# Autodesk Inventor assembly: 99535c01
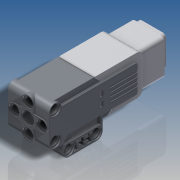
[picture p0: Inventor's stored thumbnail of the model, 180x180]
Saved by Autodesk Inventor 2016 SP2 (Build 200236200, 236)
## iProperties
Created: 2015-09-02
Part Number: 99535c01
Document SubType Name: Assembly
Designer: D. Kohfeld
Mass: 14.5508 g
Surface Area: 210.492 cm^2
Volume: 13.7272 cm^3
Density: 1.06 g/cm^3
Author: D. Kohfeld
## Documents named in this file (5)
- A:\LEGO Pieces\EV3\99535c01.iam
- A:\LEGO Pieces\EV3\99534-White.ipt
- A:\LEGO Pieces\EV3\54732b-LtBluishGray.ipt
- A:\LEGO Pieces\EV3\99542-MilkyWhite.ipt
- A:\LEGO Pieces\EV3\99535-LtBluishGray.ipt
## Components (4 placed, 4 different names)
1. 99534-White:1 — Mate:1, Mate:2, Flush:1, Flush:2, Flush:3, Mate:3
2. 54732b-LtBluishGray:1 — Mate:1, Mate:2, Flush:1
3. 99542-MilkyWhite:1 — Insert:1
4. 99535-LtBluishGray:1 — Flush:2, Flush:3, Mate:3, Insert:1
## Relationships (7: Mate 3, Flush 3, Insert 1)
- Mate:1: 99534-White:1 ↔ 54732b-LtBluishGray:1
- Mate:2: 99534-White:1 ↔ 54732b-LtBluishGray:1
- Flush:1: 99534-White:1 ↔ 54732b-LtBluishGray:1
- Flush:2: 99534-White:1 ↔ 99535-LtBluishGray:1
- Flush:3: 99534-White:1 ↔ 99535-LtBluishGray:1
- Mate:3: 99534-White:1 ↔ 99535-LtBluishGray:1
- Insert:1: 99542-MilkyWhite:1 ↔ 99535-LtBluishGray:1
